# Autodesk Inventor assembly: enclosure
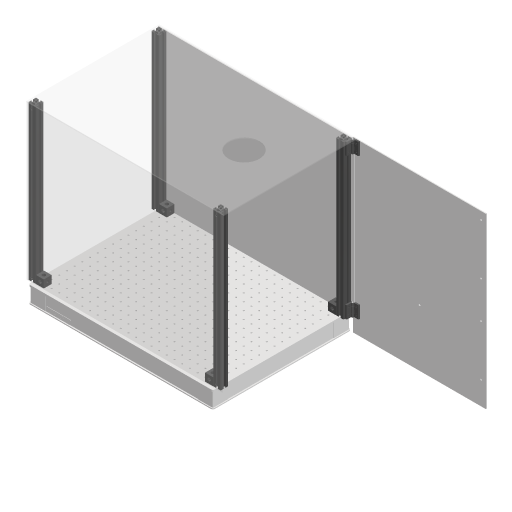
[picture p0: Inventor's stored thumbnail of the model, 512x512]
Saved by Autodesk Inventor 2023 (Build 270158000, 158)
## iProperties
Created: 2024-06-07
Part Number: enclosure
Document SubType Name: Assembly
Designer: nvladi
Author: nvladi
## Documents named in this file (9)
- C:\Users\Public\github\benchtop-hardware\Benchtop\CAD-model-Inventor\mesoSPIM\enclosure\enclosure.iam
- C:\Users\Public\github\benchtop-hardware\Benchtop\CAD-model-Inventor\library\Thorlabs\extrusions\XE25L500_M.ipt
- C:\Users\Public\github\benchtop-hardware\Benchtop\CAD-model-Inventor\library\Thorlabs\breadboards\PBG52522.ipt
- C:\Users\Public\github\benchtop-hardware\Benchtop\CAD-model-Inventor\library\Thorlabs\extrusions\RM1G.ipt
- C:\Users\Public\github\benchtop-hardware\Benchtop\CAD-model-Inventor\library\Thorlabs\extrusions\XE25H.ipt
- C:\Users\Public\github\benchtop-hardware\Benchtop\custom-parts\enclosure\front_door.ipt
- C:\Users\Public\github\benchtop-hardware\Benchtop\custom-parts\enclosure\left_wall.ipt
- C:\Users\Public\github\benchtop-hardware\Benchtop\custom-parts\enclosure\right_wall.ipt
- C:\Users\Public\github\benchtop-hardware\Benchtop\custom-parts\enclosure\top-ventilation-hole-100mm.ipt
## Components (15 placed, 8 different names)
1. XE25L500_M:1 — Mate:2, Flush:3, Flush:4, Angle:4, Flush:15
2. XE25L500_M:2 — Mate:1, Flush:1, Flush:2, Flush:13
3. XE25L500_M:3 — Mate:3, Flush:5, Flush:6, Angle:1, Mate:7, Insert:6
4. XE25L500_M:4 — Mate:4, Flush:7, Flush:8, Angle:2, Mate:5, Flush:9, Flush:10, Mate:6, Flush:11, Flush:12, Angle:3, Flush:14, Mate:9
5. PBG52522:1 — Insert:1, Insert:2, Insert:3, Insert:4, Angle:1, Angle:2, Mate:8, Angle:4, Angle:5
6. RM1G:1 — Mate:1, Flush:1, Flush:2, Insert:3
7. RM1G:2 — Mate:2, Flush:3, Flush:4, Insert:4
8. RM1G:3 — Mate:3, Flush:5, Flush:6, Insert:2
9. RM1G:4 — Mate:4, Flush:7, Flush:8, Insert:1
10. XE25H:1 — Mate:5, Flush:9, Flush:10, Insert:5
11. XE25H:2 — Mate:6, Flush:11, Flush:12
12. front_door:1 — Insert:5, Angle:3
13. left_wall:1 — Mate:7, Flush:13, Mate:8
14. right_wall:1 — Flush:14, Mate:9, Flush:15
15. top-ventilation-hole-100mm:1 — Insert:6, Angle:5
## Relationships (35: Flush 15, Mate 9, Insert 6, Angle 5)
- Mate:1: XE25L500_M:2 ↔ RM1G:1
- Flush:1: XE25L500_M:2 ↔ RM1G:1
- Flush:2: XE25L500_M:2 ↔ RM1G:1
- Mate:2: XE25L500_M:1 ↔ RM1G:2
- Flush:3: XE25L500_M:1 ↔ RM1G:2
- Flush:4: XE25L500_M:1 ↔ RM1G:2
- Mate:3: XE25L500_M:3 ↔ RM1G:3
- Flush:5: XE25L500_M:3 ↔ RM1G:3
- Flush:6: XE25L500_M:3 ↔ RM1G:3
- Mate:4: XE25L500_M:4 ↔ RM1G:4
- Flush:7: XE25L500_M:4 ↔ RM1G:4
- Flush:8: XE25L500_M:4 ↔ RM1G:4
- Insert:1: PBG52522:1 ↔ RM1G:4
- Insert:2: PBG52522:1 ↔ RM1G:3
- Insert:3: PBG52522:1 ↔ RM1G:1
- Insert:4: PBG52522:1 ↔ RM1G:2
- Angle:1 (0 deg): XE25L500_M:3 ↔ PBG52522:1
- Angle:2 (0 deg): XE25L500_M:4 ↔ PBG52522:1
- Mate:5: XE25L500_M:4 ↔ XE25H:1
- Flush:9 (5 mm): XE25L500_M:4 ↔ XE25H:1
- Flush:10: XE25L500_M:4 ↔ XE25H:1
- Mate:6: XE25L500_M:4 ↔ XE25H:2
- Flush:11 (5 mm): XE25L500_M:4 ↔ XE25H:2
- Flush:12: XE25L500_M:4 ↔ XE25H:2
- Insert:5: XE25H:1 ↔ front_door:1
- Angle:3 (180 deg): XE25L500_M:4 ↔ front_door:1
- Mate:7: XE25L500_M:3 ↔ left_wall:1
- Flush:13 (-3 mm): XE25L500_M:2 ↔ left_wall:1
- Mate:8: PBG52522:1 ↔ left_wall:1
- Flush:14: XE25L500_M:4 ↔ right_wall:1
- Mate:9: XE25L500_M:4 ↔ right_wall:1
- Angle:4 (0 deg): XE25L500_M:1 ↔ PBG52522:1
- Flush:15 (-3 mm): XE25L500_M:1 ↔ right_wall:1
- Insert:6: XE25L500_M:3 ↔ top-ventilation-hole-100mm:1
- Angle:5 (0 deg): PBG52522:1 ↔ top-ventilation-hole-100mm:1
